# Autodesk Inventor assembly: montagem
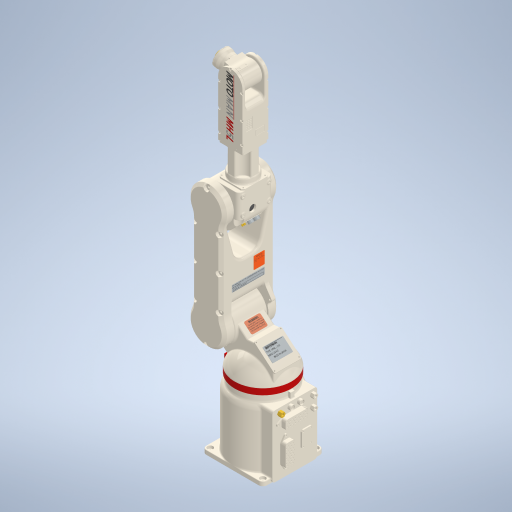
[picture p0: Inventor's stored thumbnail of the model, 512x512]
Saved by Autodesk Inventor 2023 (Build 270158000, 158)
## iProperties
Created: 2022-09-28
Part Number: montagem
Document SubType Name: Assembly
Designer: kleber
Author: kleber
## Documents named in this file (2)
- C:\Users\klebe\OneDrive\Documents\GitHub\Sala-braquiterapia\Sala de Braquiterapia\Inventor\montagem.iam
- C:\Users\klebe\OneDrive\Documents\GitHub\Sala-braquiterapia\Sala de Braquiterapia\Inventor\MH5Lmontagem oficial.iam
## Components (1 placed, 1 different names)
1. MH5Lmontagem oficial:1 [sub-assembly] — Mate:1
## Relationships (1: Mate 1)
- Mate:1: MH5Lmontagem oficial:1
